# Autodesk Inventor assembly: 001_ring_dntmove
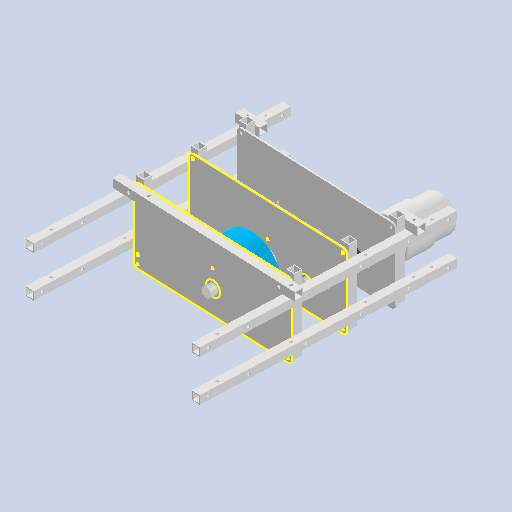
[picture p0: Inventor's stored thumbnail of the model, 512x512]
Saved by Autodesk Inventor 2025.1 (Build 291241000, 241)
## iProperties
Created: 2024-10-03
Part Number: 001_ring_dntmove
Document SubType Name: Assembly
Designer: yuki0520
Author: yuki0520
## Documents named in this file (16)
- C:\Users\yuki0520\OneDrive\ドキュメント\Inventor\2025_nhk\tanaka\nageru\smallring\001_ring_shita.iam
- C:\Users\yuki0520\OneDrive\ドキュメント\Inventor\2025_nhk\tanaka\nageru\inventorパーツリスト\モーター\775\RS-775GM.ipt
- C:\Users\yuki0520\OneDrive\ドキュメント\Inventor\2025_nhk\tanaka\nageru\inventorパーツリスト\モーター\775\RS-775GM_004GH_sn.ipt
- C:\Users\yuki0520\OneDrive\ドキュメント\Inventor\2025_nhk\tanaka\nageru\pakuriz\TH22_Bar_motor_roller_sn.ipt
- C:\Users\yuki0520\OneDrive\ドキュメント\Inventor\2025_nhk\tanaka\nageru\pakuriz\kaku_1010_120.ipt
- C:\Users\yuki0520\OneDrive\ドキュメント\Inventor\2025_nhk\tanaka\nageru\pakuriz\bear_12_18.ipt
- C:\Users\yuki0520\OneDrive\ドキュメント\Inventor\2025_nhk\tanaka\nageru\smallring\small_tire.ipt
- C:\Users\yuki0520\OneDrive\ドキュメント\Inventor\2025_nhk\tanaka\nageru\smallring\small_tire_fixer.ipt
- C:\Users\yuki0520\OneDrive\ドキュメント\Inventor\2025_nhk\tanaka\nageru\smallring\small_bar_roller.ipt
- C:\Users\yuki0520\OneDrive\ドキュメント\Inventor\2025_nhk\tanaka\nageru\smallring\small_gear_motor_48.iam
- C:\Users\yuki0520\OneDrive\ドキュメント\Inventor\2025_nhk\tanaka\nageru\smallring\small_kaku_1010_bridge.ipt
- C:\Users\yuki0520\OneDrive\ドキュメント\Inventor\2025_nhk\tanaka\nageru\smallring\small_kaku_1010_santen.ipt
- C:\Users\yuki0520\OneDrive\ドキュメント\Inventor\2025_nhk\tanaka\nageru\smallring\small_kaku_1010_200.ipt
- C:\Users\yuki0520\OneDrive\ドキュメント\Inventor\2025_nhk\tanaka\nageru\smallring\small_plate_shita_motor.ipt
- C:\Users\yuki0520\OneDrive\ドキュメント\Inventor\2025_nhk\tanaka\nageru\smallring\small_plate_shita_middle.ipt
- C:\Users\yuki0520\OneDrive\ドキュメント\Inventor\2025_nhk\tanaka\nageru\smallring\small_plate_shita_nomotor.ipt
## Components (28 placed, 15 different names)
1. RS-775GM:1 — メイト:4, 正接:1
2. RS-775GM_004GH_sn:1 — メイト:4, 正接:1, メイト:5, メイト:7, 挿入:110, 挿入:111
3. TH22_Bar_motor_roller_sn:1 — メイト:5, メイト:7, メイト:28, メイト:29
4. kaku_1010_120:1 — 挿入:83, 挿入:89, 挿入:96, 挿入:112
5. kaku_1010_120:2 — 挿入:86, 挿入:92, 挿入:107
6. kaku_1010_120:3 — 挿入:81, 挿入:87, メイト:80, 挿入:105, 挿入:106, メイト:86
7. kaku_1010_120:4 — 挿入:85, 挿入:91, 挿入:103
8. bear_12_18:1 — メイト:33, メイト:84
9. bear_12_18:2 — メイト:35, メイト:85, メイト:87
10. kaku_1010_120:5 — 挿入:82, 挿入:88, 挿入:102, 挿入:104
11. kaku_1010_120:6 — 挿入:84, 挿入:90, 挿入:95, 挿入:108, 挿入:109
12. bear_12_18:3 — メイト:31
13. small_tire:1 — 挿入:25, 挿入:26, メイト:8, 挿入:39, 挿入:40
14. small_tire_fixer:1 — 挿入:25, 挿入:26, メイト:9
15. small_bar_roller:1 — メイト:8, メイト:9, メイト:27, メイト:30, メイト:31, メイト:33, メイト:35, メイト:38, メイト:81, メイト:82, メイト:87
16. small_gear_motor_48:1 [sub-assembly] — メイト:27, メイト:28, メイト:29, メイト:38
17. small_tire_fixer:2 — 挿入:39, 挿入:40, メイト:30
18. small_kaku_1010_bridge:1 — 挿入:93, 挿入:94, メイト:80
19. small_kaku_1010_santen:1 — 挿入:80, 挿入:95
20. small_kaku_1010_santen:2 — 挿入:71, 挿入:96
21. small_kaku_1010_200:1 — 挿入:71, 挿入:81, 挿入:82, 挿入:83, 挿入:94
22. small_kaku_1010_200:2 — 挿入:87, 挿入:88, 挿入:89
23. small_kaku_1010_200:3 — 挿入:90, 挿入:91, 挿入:92
24. small_kaku_1010_200:4 — 挿入:80, 挿入:84, 挿入:85, 挿入:86, 挿入:93
25. small_plate_shita_motor:1 — メイト:85, 挿入:108, 挿入:109, 挿入:110, 挿入:111, 挿入:112
26. small_plate_shita_middle:1 — 挿入:102, 挿入:103, 挿入:104, メイト:84
27. small_plate_shita_nomotor:1 — 挿入:105, 挿入:106, 挿入:107, メイト:81, メイト:83
28. bear_12_18:4 — メイト:82, メイト:83
## Relationships (55: Insert 33, Mate 21, Tangent 1)
- メイト:4 [Mate]: RS-775GM:1 ↔ RS-775GM_004GH_sn:1
- 正接:1 [Tangent]: RS-775GM:1 ↔ RS-775GM_004GH_sn:1
- メイト:5 [Mate]: RS-775GM_004GH_sn:1 ↔ TH22_Bar_motor_roller_sn:1
- メイト:7 [Mate]: RS-775GM_004GH_sn:1 ↔ TH22_Bar_motor_roller_sn:1
- 挿入:25 [Insert]: small_tire:1 ↔ small_tire_fixer:1
- 挿入:26 [Insert]: small_tire:1 ↔ small_tire_fixer:1
- メイト:8 [Mate]: small_tire:1 ↔ small_bar_roller:1
- メイト:9 [Mate]: small_tire_fixer:1 ↔ small_bar_roller:1
- メイト:27 [Mate]: small_bar_roller:1 ↔ small_gear_motor_48:1
- メイト:28 [Mate]: TH22_Bar_motor_roller_sn:1 ↔ small_gear_motor_48:1
- メイト:29 [Mate]: TH22_Bar_motor_roller_sn:1 ↔ small_gear_motor_48:1
- 挿入:39 [Insert]: small_tire:1 ↔ small_tire_fixer:2
- 挿入:40 [Insert]: small_tire:1 ↔ small_tire_fixer:2
- メイト:30 [Mate]: small_bar_roller:1 ↔ small_tire_fixer:2
- メイト:31 [Mate]: bear_12_18:3 ↔ small_bar_roller:1
- メイト:33 [Mate]: bear_12_18:1 ↔ small_bar_roller:1
- メイト:35 [Mate]: bear_12_18:2 ↔ small_bar_roller:1
- メイト:38 [Mate]: small_bar_roller:1 ↔ small_gear_motor_48:1
- 挿入:71 [Insert]: small_kaku_1010_santen:2 ↔ small_kaku_1010_200:1
- 挿入:80 [Insert]: small_kaku_1010_santen:1 ↔ small_kaku_1010_200:4
- 挿入:81 [Insert]: kaku_1010_120:3 ↔ small_kaku_1010_200:1
- 挿入:82 [Insert]: kaku_1010_120:5 ↔ small_kaku_1010_200:1
- 挿入:83 [Insert]: kaku_1010_120:1 ↔ small_kaku_1010_200:1
- 挿入:84 [Insert]: kaku_1010_120:6 ↔ small_kaku_1010_200:4
- 挿入:85 [Insert]: kaku_1010_120:4 ↔ small_kaku_1010_200:4
- 挿入:86 [Insert]: kaku_1010_120:2 ↔ small_kaku_1010_200:4
- 挿入:87 [Insert]: kaku_1010_120:3 ↔ small_kaku_1010_200:2
- 挿入:88 [Insert]: kaku_1010_120:5 ↔ small_kaku_1010_200:2
- 挿入:89 [Insert]: kaku_1010_120:1 ↔ small_kaku_1010_200:2
- 挿入:90 [Insert]: kaku_1010_120:6 ↔ small_kaku_1010_200:3
- 挿入:91 [Insert]: kaku_1010_120:4 ↔ small_kaku_1010_200:3
- 挿入:92 [Insert]: kaku_1010_120:2 ↔ small_kaku_1010_200:3
- 挿入:93 [Insert]: small_kaku_1010_bridge:1 ↔ small_kaku_1010_200:4
- 挿入:94 [Insert]: small_kaku_1010_bridge:1 ↔ small_kaku_1010_200:1
- メイト:80 [Mate]: kaku_1010_120:3 ↔ small_kaku_1010_bridge:1
- 挿入:95 [Insert]: kaku_1010_120:6 ↔ small_kaku_1010_santen:1
- 挿入:96 [Insert]: kaku_1010_120:1 ↔ small_kaku_1010_santen:2
- 挿入:102 [Insert]: kaku_1010_120:5 ↔ small_plate_shita_middle:1
- 挿入:103 [Insert]: kaku_1010_120:4 ↔ small_plate_shita_middle:1
- 挿入:104 [Insert]: kaku_1010_120:5 ↔ small_plate_shita_middle:1
- 挿入:105 [Insert]: kaku_1010_120:3 ↔ small_plate_shita_nomotor:1
- 挿入:106 [Insert]: kaku_1010_120:3 ↔ small_plate_shita_nomotor:1
- 挿入:107 [Insert]: kaku_1010_120:2 ↔ small_plate_shita_nomotor:1
- メイト:81 [Mate]: small_bar_roller:1 ↔ small_plate_shita_nomotor:1
- メイト:82 [Mate]: small_bar_roller:1 ↔ bear_12_18:4
- メイト:83 [Mate]: small_plate_shita_nomotor:1 ↔ bear_12_18:4
- メイト:84 [Mate]: bear_12_18:1 ↔ small_plate_shita_middle:1
- メイト:85 [Mate]: bear_12_18:2 ↔ small_plate_shita_motor:1
- メイト:86 [Mate]: kaku_1010_120:3
- 挿入:108 [Insert]: kaku_1010_120:6 ↔ small_plate_shita_motor:1
- 挿入:109 [Insert]: kaku_1010_120:6 ↔ small_plate_shita_motor:1
- 挿入:110 [Insert]: RS-775GM_004GH_sn:1 ↔ small_plate_shita_motor:1
- 挿入:111 [Insert]: RS-775GM_004GH_sn:1 ↔ small_plate_shita_motor:1
- 挿入:112 [Insert]: kaku_1010_120:1 ↔ small_plate_shita_motor:1
- メイト:87 [Mate]: bear_12_18:2 ↔ small_bar_roller:1
